# Autodesk Inventor assembly: Cutting machine assembly
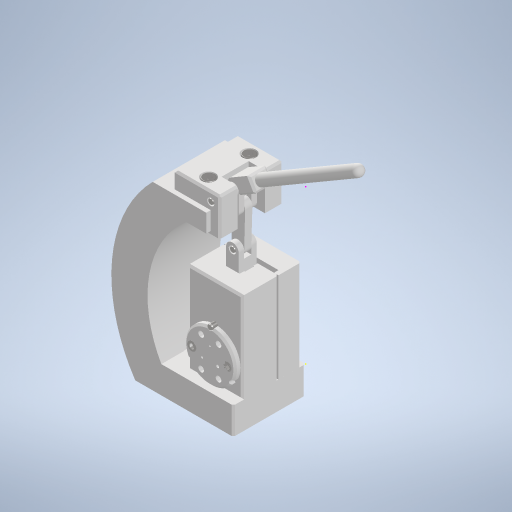
[picture p0: Inventor's stored thumbnail of the model, 512x512]
Saved by Autodesk Inventor 2023.2 (Build 272271030, 271C)
## iProperties
Created: 2023-02-12
Part Number: Cutting machine assembly
Document SubType Name: Assembly
Designer: Ayush
Author: Ayush
## Documents named in this file (17)
- F:\MS\SRH study\CAD projects\Bonus Assignment\Cutting machine assembly.iam
- F:\MS\SRH study\CAD projects\Bonus Assignment\Schneidführung.ipt
- F:\MS\SRH study\CAD projects\Bonus Assignment\Schneidführungsdeckel.ipt
- F:\MS\SRH study\CAD projects\Bonus Assignment\Schneidtrommel.ipt
- F:\MS\SRH study\CAD projects\Bonus Assignment\Schneidstempel.ipt
- F:\MS\SRH study\CAD projects\Bonus Assignment\Gestell.ipt
- F:\MS\SRH study\CAD projects\Bonus Assignment\Hebel.ipt
- F:\MS\SRH study\CAD projects\Bonus Assignment\Lager.ipt
- F:\MS\SRH study\CAD projects\Bonus Assignment\Kniehebel.ipt
- C:\Users\Ayush\Documents\Inventor\Content Center Files\R2023\en-US\DIN 912\DIN 912 - M8 x 1.25 x 30 x 26.875.ipt
- C:\Users\Ayush\Documents\Inventor\Content Center Files\R2023\en-US\DIN 912\DIN 912 - M8 x 1.25 x 20 x 16.875.ipt
- C:\Users\Ayush\Documents\Inventor\Content Center Files\R2023\en-US\DIN 912\DIN 912 - M6 x 1 x 25 x 22.5.ipt
- C:\Users\Ayush\Documents\Inventor\Content Center Files\R2023\en-US\ISO 2338(4)\ISO 2338 - 6 m6 x 20 - ADIN EN.ipt
- C:\Users\Ayush\Documents\Inventor\Content Center Files\R2023\en-US\ISO 2338(4)\ISO 2338 - 6 m6 x 70 - ADIN EN.ipt
- C:\Users\Ayush\Documents\Inventor\Content Center Files\R2023\en-US\ISO 2338(4)\ISO 2338 - 6 m6 x 16 - ADIN EN.ipt
- C:\Users\Ayush\Documents\Inventor\Content Center Files\R2023\en-US\DIN 912\DIN 912 - M6 x 1 x 16 x 13.5.ipt
- F:\MS\SRH study\CAD projects\Bonus Assignment\Griff.ipt
## Components (27 placed, 16 different names)
1. Schneidführung:1 — Mate:1, Flush:1, Flush:2, Mate:2, Mate:3, Mate:4, Mate:6, Flush:4, Mate:16, Mate:21, Insert:13
2. Schneidführungsdeckel:1 — Mate:1, Flush:1, Flush:2, Flush:5, Insert:7, Insert:8, Insert:9, Insert:10, Insert:11, Insert:12
3. Schneidtrommel:1 — Mate:2, Mate:3, Mate:4, Mate:22, Insert:14
4. Gestell:1 — Mate:6, Flush:4, Flush:5, Mate:9, Flush:6, Flush:7, Insert:1, Insert:2, Insert:3, Insert:4
5. Hebel:1 — Mate:12, Mate:13, Mate:14, Mate:15, Mate:19
6. Lager:1 — Mate:9, Flush:6, Flush:7, Mate:10, Mate:17, Insert:5, Insert:6, Mate:20, Flush:9
7. Kniehebel:1 — Mate:10, Mate:12, Mate:13, Mate:17, Flush:8, Insert:15
8. Schneidstempel:1 — Mate:14, Mate:15, Mate:16, Mate:23, Flush:10
9. DIN 912 - replaced by DIN EN ISO 4762 M8 x 30:1 — Insert:4
10. DIN 912 - replaced by DIN EN ISO 4762 M8 x 30:2 — Insert:2
11. DIN 912 - replaced by DIN EN ISO 4762 M8 x 30:3 — Insert:3
12. DIN 912 - replaced by DIN EN ISO 4762 M8 x 30:4 — Insert:1
13. DIN 912 - replaced by DIN EN ISO 4762 M8 x 20:1 — Insert:5
14. DIN 912 - replaced by DIN EN ISO 4762 M8 x 20:2 — Insert:6
15. DIN 912 - replaced by DIN EN ISO 4762 M6 x 25:1 — Insert:8
16. DIN 912 - replaced by DIN EN ISO 4762 M6 x 25:2 — Insert:7
17. DIN 912 - replaced by DIN EN ISO 4762 M6 x 25:3 — Insert:9
18. DIN 912 - replaced by DIN EN ISO 4762 M6 x 25:4 — Insert:10
19. DIN 912 - replaced by DIN EN ISO 4762 M6 x 25:5 — Insert:12
20. DIN 912 - replaced by DIN EN ISO 4762 M6 x 25:6 — Insert:11
21. DIN EN 22338 A - withdrawn 6 m6 x 20 - A:1 — Mate:19, Flush:8
22. DIN EN 22338 A - withdrawn 6 m6 x 70 - A:1 — Mate:20, Flush:9
23. DIN EN 22338 A - withdrawn 6 m6 x 16 - A:1 — Mate:21, Mate:22
24. DIN 912 - replaced by DIN EN ISO 4762 M6 x 16:1 — Insert:13
25. DIN 912 - replaced by DIN EN ISO 4762 M6 x 16:2 — Insert:14
26. Griff:1 — Insert:15
27. DIN EN 22338 A - withdrawn 6 m6 x 20 - A:2 — Mate:23, Flush:10
## Relationships (42: Mate 18, Insert 15, Flush 9)
- Mate:1: Schneidführung:1 ↔ Schneidführungsdeckel:1
- Flush:1: Schneidführung:1 ↔ Schneidführungsdeckel:1
- Flush:2: Schneidführung:1 ↔ Schneidführungsdeckel:1
- Mate:2: Schneidführung:1 ↔ Schneidtrommel:1
- Mate:3: Schneidführung:1 ↔ Schneidtrommel:1
- Mate:4: Schneidführung:1 ↔ Schneidtrommel:1
- Mate:6: Schneidführung:1 ↔ Gestell:1
- Flush:4: Schneidführung:1 ↔ Gestell:1
- Flush:5: Schneidführungsdeckel:1 ↔ Gestell:1
- Mate:9: Gestell:1 ↔ Lager:1
- Flush:6: Gestell:1 ↔ Lager:1
- Flush:7: Gestell:1 ↔ Lager:1
- Mate:10: Lager:1 ↔ Kniehebel:1
- Mate:12: Hebel:1 ↔ Kniehebel:1
- Mate:13: Hebel:1 ↔ Kniehebel:1
- Mate:14: Hebel:1 ↔ Schneidstempel:1
- Mate:15: Hebel:1 ↔ Schneidstempel:1
- Mate:16: Schneidführung:1 ↔ Schneidstempel:1
- Mate:17: Lager:1 ↔ Kniehebel:1
- Insert:1: Gestell:1 ↔ DIN 912 - replaced by DIN EN ISO 4762 M8 x 30:4
- Insert:2: Gestell:1 ↔ DIN 912 - replaced by DIN EN ISO 4762 M8 x 30:2
- Insert:3: Gestell:1 ↔ DIN 912 - replaced by DIN EN ISO 4762 M8 x 30:3
- Insert:4: Gestell:1 ↔ DIN 912 - replaced by DIN EN ISO 4762 M8 x 30:1
- Insert:5: Lager:1 ↔ DIN 912 - replaced by DIN EN ISO 4762 M8 x 20:1
- Insert:6: Lager:1 ↔ DIN 912 - replaced by DIN EN ISO 4762 M8 x 20:2
- Insert:7: Schneidführungsdeckel:1 ↔ DIN 912 - replaced by DIN EN ISO 4762 M6 x 25:2
- Insert:8: Schneidführungsdeckel:1 ↔ DIN 912 - replaced by DIN EN ISO 4762 M6 x 25:1
- Insert:9: Schneidführungsdeckel:1 ↔ DIN 912 - replaced by DIN EN ISO 4762 M6 x 25:3
- Insert:10: Schneidführungsdeckel:1 ↔ DIN 912 - replaced by DIN EN ISO 4762 M6 x 25:4
- Insert:11: Schneidführungsdeckel:1 ↔ DIN 912 - replaced by DIN EN ISO 4762 M6 x 25:6
- Insert:12: Schneidführungsdeckel:1 ↔ DIN 912 - replaced by DIN EN ISO 4762 M6 x 25:5
- Mate:19: Hebel:1 ↔ DIN EN 22338 A - withdrawn 6 m6 x 20 - A:1
- Flush:8: Kniehebel:1 ↔ DIN EN 22338 A - withdrawn 6 m6 x 20 - A:1
- Mate:20: Lager:1 ↔ DIN EN 22338 A - withdrawn 6 m6 x 70 - A:1
- Flush:9: Lager:1 ↔ DIN EN 22338 A - withdrawn 6 m6 x 70 - A:1
- Mate:21: Schneidführung:1 ↔ DIN EN 22338 A - withdrawn 6 m6 x 16 - A:1
- Mate:22: Schneidtrommel:1 ↔ DIN EN 22338 A - withdrawn 6 m6 x 16 - A:1
- Insert:13: Schneidführung:1 ↔ DIN 912 - replaced by DIN EN ISO 4762 M6 x 16:1
- Insert:14: Schneidtrommel:1 ↔ DIN 912 - replaced by DIN EN ISO 4762 M6 x 16:2
- Insert:15: Kniehebel:1 ↔ Griff:1
- Mate:23: Schneidstempel:1 ↔ DIN EN 22338 A - withdrawn 6 m6 x 20 - A:2
- Flush:10: Schneidstempel:1 ↔ DIN EN 22338 A - withdrawn 6 m6 x 20 - A:2
